# Autodesk Inventor assembly: SHOCK ABSORBER2
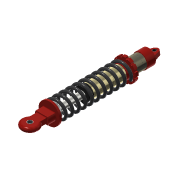
[picture p0: Inventor's stored thumbnail of the model, 180x180]
Saved by Autodesk Inventor 2019 (Build 230136000, 136)
## iProperties
Created: 2023-06-18
Part Number: SHOCK ABSORBER2
Document SubType Name: Assembly
Designer: Fransic
Author: Fransic
## Documents named in this file (14)
- C:\Users\Fransic\Documents\Inventor\Shock Absorber\SHOCK ABSORBER2.iam
- C:\Users\Fransic\Documents\Inventor\Shock Absorber\STRUT MOUNT.ipt
- C:\Users\Fransic\Documents\Inventor\Shock Absorber\TOP STRUT MOUNT.ipt
- C:\Users\Fransic\Documents\Inventor\Shock Absorber\ADJUSTABLE DISC.ipt
- C:\Users\Fransic\Documents\Inventor\Shock Absorber\SPRING SUPPORT.ipt
- C:\Users\Fransic\Documents\Inventor\Shock Absorber\PISTON GUIDE.ipt
- C:\Users\Fransic\Documents\Inventor\Shock Absorber\BASE VALVE.ipt
- C:\Users\Fransic\Documents\Inventor\Shock Absorber\OIL RING.ipt
- C:\Users\Fransic\Documents\Inventor\Shock Absorber\PISTON.ipt
- C:\Users\Fransic\Documents\Inventor\Shock Absorber\COIL SPRING.ipt
- C:\Users\Fransic\Documents\Inventor\Shock Absorber\STRUTMOUNT  PART.ipt
- C:\Users\Fransic\Documents\Inventor\Shock Absorber\2 STRUTMOUNT  PART.ipt
- C:\Users\Fransic\Documents\Inventor\Shock Absorber\RUBBER.ipt
- C:\Users\Fransic\Documents\Inventor\Shock Absorber\RUBBER2.ipt
## Components (13 placed, 13 different names)
1. STRUT MOUNT:1 — Mate:1, SPRING DRIVE, Mate:5, Mate:6, Mate:14, Flush:3, Mate:16, Mate:18, Rotation:1
2. TOP STRUT MOUNT:1 — Mate:1, Mate:2, Mate:3, Mate:7, Mate:8, Mate:9, Mate:10, Mate:19, Mate:20, Rotation:1
3. ADJUSTABLE DISC:1 — Mate:2, SPRING DRIVE, Mate:3, Flush:2
4. SPRING SUPPORT:1 — Mate:5, Mate:6, Flush:1
5. PISTON GUIDE:1 — Mate:7, Mate:8, Mate:13
6. BASE VALVE:1 — Mate:9, Mate:10, Mate:11, Mate:12
7. OIL RING:1 — Mate:11, Mate:12
8. PISTON:1 — Mate:13, Mate:14, Mate:15
9. COIL SPRING:1 — Flush:1, Flush:2, Flush:3, Mate:15
10. STRUTMOUNT  PART:1 — Mate:16, Mate:18, Mate:24, Mate:25
11. 2 STRUTMOUNT  PART:1 — Mate:19, Mate:20, Mate:22, Mate:23
12. RUBBER:2 — Mate:22, Mate:23
13. RUBBER2:1 — Mate:24, Mate:25
## Relationships (27: Mate 23, Flush 3, RelateRotation 1)
- Mate:1: STRUT MOUNT:1 ↔ TOP STRUT MOUNT:1
- Mate:2: TOP STRUT MOUNT:1 ↔ ADJUSTABLE DISC:1
- SPRING DRIVE [Mate] (300 mm): STRUT MOUNT:1 ↔ ADJUSTABLE DISC:1
- Mate:5: STRUT MOUNT:1 ↔ SPRING SUPPORT:1
- Mate:6: STRUT MOUNT:1 ↔ SPRING SUPPORT:1
- Mate:7: TOP STRUT MOUNT:1 ↔ PISTON GUIDE:1
- Mate:8: TOP STRUT MOUNT:1 ↔ PISTON GUIDE:1
- Mate:9: TOP STRUT MOUNT:1 ↔ BASE VALVE:1
- Mate:10: TOP STRUT MOUNT:1 ↔ BASE VALVE:1
- Mate:11: BASE VALVE:1 ↔ OIL RING:1
- Mate:12: BASE VALVE:1 ↔ OIL RING:1
- Mate:13: PISTON GUIDE:1 ↔ PISTON:1
- Mate:14: STRUT MOUNT:1 ↔ PISTON:1
- Flush:1: SPRING SUPPORT:1 ↔ COIL SPRING:1
- Mate:3 (12 mm): TOP STRUT MOUNT:1 ↔ ADJUSTABLE DISC:1
- Flush:2: ADJUSTABLE DISC:1 ↔ COIL SPRING:1
- Flush:3: STRUT MOUNT:1 ↔ COIL SPRING:1
- Mate:15: PISTON:1 ↔ COIL SPRING:1
- Mate:16: STRUT MOUNT:1 ↔ STRUTMOUNT  PART:1
- Mate:18: STRUT MOUNT:1 ↔ STRUTMOUNT  PART:1
- Mate:19: TOP STRUT MOUNT:1 ↔ 2 STRUTMOUNT  PART:1
- Mate:20: TOP STRUT MOUNT:1 ↔ 2 STRUTMOUNT  PART:1
- Mate:22: 2 STRUTMOUNT  PART:1 ↔ RUBBER:2
- Mate:23: 2 STRUTMOUNT  PART:1 ↔ RUBBER:2
- Mate:24: STRUTMOUNT  PART:1 ↔ RUBBER2:1
- Mate:25: STRUTMOUNT  PART:1 ↔ RUBBER2:1
- Rotation:1 [RelateRotation] (1 ul): STRUT MOUNT:1 ↔ TOP STRUT MOUNT:1
